# Autodesk Inventor assembly: RPR-900
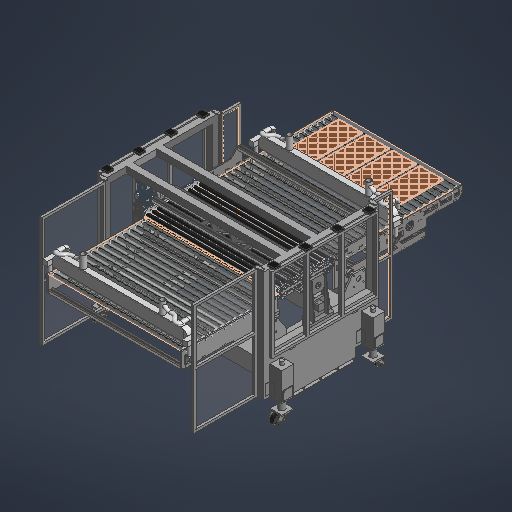
[picture p0: Inventor's stored thumbnail of the model, 512x512]
Saved by Autodesk Inventor 2025 (Build 290162000, 162)
## iProperties
Created: 2024-05-07
Part Number: RPR-900
Document SubType Name: Assembly
Designer: zulet
Author: zulet
## Documents named in this file (9)
- D:\UNAL\2024-1S\APM\Digital Factory\Ceramic Press\SACMI RPR 900\RPR-900.iam
- D:\UNAL\2024-1S\APM\Digital Factory\Ceramic Press\SACMI RPR 900\RPR-900 BASE.ipt
- D:\UNAL\2024-1S\APM\Digital Factory\Conveyor System\CONVEYOR ROLLER\CR-1640.ipt
- D:\UNAL\2024-1S\APM\Digital Factory\Conveyor System\CONVEYOR ROLLER.ipt
- D:\UNAL\2024-1S\APM\Digital Factory\Conveyor System\CONVEYOR ROLLER\CR-1580.ipt
- D:\UNAL\2024-1S\APM\Digital Factory\Three Phased Motors\tm71-2m-b5\tm71-2m-b5.ipt
- D:\UNAL\2024-1S\APM\Digital Factory\Worm Gear Boxes\s_50\s_50.ipt
- D:\UNAL\2024-1S\APM\Digital Factory\Ceramic Press\SACMI RPR 900\RPR-900 UNIVERSAL TIPPER.ipt
- D:\UNAL\2024-1S\APM\Digital Factory\TILE 30X60.ipt
## Components (65 placed, 7 different names)
1. RPR-900 BASE:1 — Mate:1, Flush:1, Mate:2, Flush:2, Mate:3, Flush:3, Mate:5, Flush:7, Flush:8, Rotational:1, Flush:10, Angle:1
2. tm71-2m-b5:1 — Mate:4, Mate:6
3. s_50:1 — Mate:4, Mate:5, Flush:7, Flush:8, Mate:6
4. RPR-900 UNIVERSAL TIPPER:1 — Rotational:1, Mate:7, Flush:9
5. CR-1580:3 — Mate:1, Flush:1
6. CR-1580:4
7. CR-1580:5
8. CR-1580:6
9. CR-1580:7
10. CR-1580:8
11. CR-1580:9
12. CR-1580:10
13. CR-1580:11
14. CR-1580:12
15. CR-1580:13
16. CR-1580:14
17. CR-1580:15
18. CR-1640:1 — Mate:2, Flush:2
19. CR-1640:17
20. CR-1640:18
21. CR-1640:19
22. CR-1640:20
23. CR-1640:21
24. CR-1640:22
25. CR-1640:2 — Mate:3, Flush:3
26. CR-1640:23
27. CR-1640:24
28. CR-1640:25
29. CR-1640:26
30. CR-1640:27
31. CR-1640:28
32. CR-1640:29
33. CR-1640:30
34. CR-1640:31
35. CR-1640:32
36. CR-1640:33
37. CR-1640:34
38. CR-1640:35
39. CR-1640:36
40. CR-1640:37 — Mate:7, Flush:9
41. CR-1640:38
42. CR-1640:39
43. CR-1640:40
44. CR-1640:41
45. CR-1640:42
46. CR-1640:43
47. CR-1640:44
48. CR-1640:45
49. CR-1640:46
50. CR-1640:47
51. CR-1640:48
52. CR-1640:49
53. CR-1640:50
54. CR-1640:51
55. CR-1640:52
56. CR-1640:53
57. CR-1640:54
58. CR-1640:55
59. CR-1640:56
60. CR-1640:57
61. CR-1640:58
62. TILE 30X60:1 — Flush:10, Angle:1
63. TILE 30X60:2
64. TILE 30X60:3
65. TILE 30X60:4
## Component patterns: (13 elements, first: CR-1580:3), (8 elements, first: CR-1640:1), (15 elements, first: CR-1640:2), (22 elements, first: CR-1640:37), (4 elements, first: TILE 30X60:1)
## Relationships (16: Mate 7, Flush 7, RevoluteJoint 1, Angle 1)
- Mate:1: RPR-900 BASE:1 ↔ CR-1580:3
- Flush:1: RPR-900 BASE:1 ↔ CR-1580:3
- Mate:2: RPR-900 BASE:1 ↔ CR-1640:1
- Flush:2: RPR-900 BASE:1 ↔ CR-1640:1
- Mate:3: RPR-900 BASE:1 ↔ CR-1640:2
- Flush:3: RPR-900 BASE:1 ↔ CR-1640:2
- Mate:4: tm71-2m-b5:1 ↔ s_50:1
- Mate:5: RPR-900 BASE:1 ↔ s_50:1
- Flush:7: RPR-900 BASE:1 ↔ s_50:1
- Flush:8: RPR-900 BASE:1 ↔ s_50:1
- Mate:6: tm71-2m-b5:1 ↔ s_50:1
- Rotational:1 [RevoluteJoint] (102 mm): RPR-900 BASE:1 ↔ RPR-900 UNIVERSAL TIPPER:1
- Mate:7: RPR-900 UNIVERSAL TIPPER:1 ↔ CR-1640:37
- Flush:9: RPR-900 UNIVERSAL TIPPER:1 ↔ CR-1640:37
- Flush:10: RPR-900 BASE:1 ↔ TILE 30X60:1
- Angle:1 (0 deg): RPR-900 BASE:1 ↔ TILE 30X60:1
